# Autodesk Inventor assembly: 810003_Radio Shield ASSY
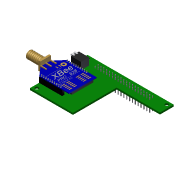
[picture p0: Inventor's stored thumbnail of the model, 180x180]
Saved by Autodesk Inventor 2015 (Build 190159000, 159)
## iProperties
Created: 2014-08-12
Part Number: 810003_Radio Shield ASSY
Document SubType Name: Assembly
Designer: david
Author: david
## Documents named in this file (6)
- C:\SharedDrive\Dropbox\FAST Robotics\Products\810003_Radio Shield\MECH\810003_Radio Shield\810003A\810003_Radio Shield ASSY.iam
- C:\SharedDrive\Dropbox\FAST Robotics\Products\810003_Radio Shield\MECH\810003_Radio Shield\810003A\MainBoard.ipt
- C:\SharedDrive\Dropbox\FAST Robotics\Products\810003_Radio Shield\MECH\810003_Radio Shield\810003A\702871018.ipt
- C:\SharedDrive\Dropbox\FAST Robotics\Library\784005_HEADER Female Socket 10pos 2mm Thru-Hole\784005_HEADER Female Socket 10pos 2mm Thru-Hole.ipt
- C:\SharedDrive\Dropbox\FAST Robotics\Library\616001_DIP Switch Side 2Pos\MECH\616001_DIP Switch Side 2Pos.ipt
- C:\SharedDrive\Dropbox\FAST Robotics\Library\363002_XBee XBP24BZ7SIT\MECH\Imported Components\User Library-XBP24BZ7SIT-004-radio\Assembly2.iam
## Components (6 placed, 5 different names)
1. MainBoard:1 — Mate:1, Flush:1, Flush:2, Flush:3, Flush:4, Flush:5, Mate:3, Mate:4, Flush:14, Flush:15, Flush:16, Flush:17
2. 702871018:1 — Mate:1, Flush:4, Flush:5
3. 784005_HEADER Female Socket 10pos 2mm Thru-Hole:1 — Flush:10, Mate:3, Mate:5, Mate:6, Flush:13, Flush:14, Flush:15, Mate:8
4. 784005_HEADER Female Socket 10pos 2mm Thru-Hole:2 — Flush:10, Flush:13, Mate:7
5. 616001_DIP Switch Side 2Pos:1 — Mate:4, Flush:16, Flush:17
6. Assembly2:1 [sub-assembly] — Mate:5, Mate:6, Mate:7, Mate:8
## Relationships (18: Flush 11, Mate 7)
- Mate:1: MainBoard:1 ↔ 702871018:1
- Flush:1: MainBoard:1
- Flush:2: MainBoard:1
- Flush:3: MainBoard:1
- Flush:4 (-13.208 mm): MainBoard:1 ↔ 702871018:1
- Flush:5 (3.048 mm): MainBoard:1 ↔ 702871018:1
- Flush:10: 784005_HEADER Female Socket 10pos 2mm Thru-Hole:1 ↔ 784005_HEADER Female Socket 10pos 2mm Thru-Hole:2
- Mate:3: MainBoard:1 ↔ 784005_HEADER Female Socket 10pos 2mm Thru-Hole:1
- Mate:4: MainBoard:1 ↔ 616001_DIP Switch Side 2Pos:1
- Mate:5: 784005_HEADER Female Socket 10pos 2mm Thru-Hole:1 ↔ Assembly2:1
- Mate:6: 784005_HEADER Female Socket 10pos 2mm Thru-Hole:1 ↔ Assembly2:1
- Flush:13: 784005_HEADER Female Socket 10pos 2mm Thru-Hole:1 ↔ 784005_HEADER Female Socket 10pos 2mm Thru-Hole:2
- Flush:14: MainBoard:1 ↔ 784005_HEADER Female Socket 10pos 2mm Thru-Hole:1
- Mate:7: 784005_HEADER Female Socket 10pos 2mm Thru-Hole:2 ↔ Assembly2:1
- Flush:15 (8.128 mm): MainBoard:1 ↔ 784005_HEADER Female Socket 10pos 2mm Thru-Hole:1
- Mate:8: 784005_HEADER Female Socket 10pos 2mm Thru-Hole:1 ↔ Assembly2:1
- Flush:16: MainBoard:1 ↔ 616001_DIP Switch Side 2Pos:1
- Flush:17 (-7.62 mm): MainBoard:1 ↔ 616001_DIP Switch Side 2Pos:1
